# Autodesk Inventor assembly: Arm_Right
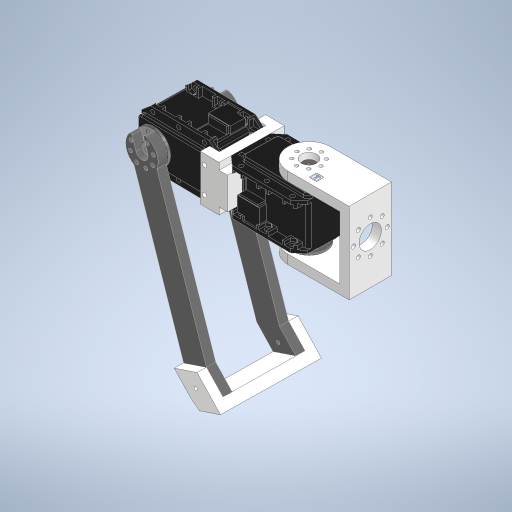
[picture p0: Inventor's stored thumbnail of the model, 512x512]
Saved by Autodesk Inventor 2024.3 (Build 283343000, 343)
## iProperties
Created: 2024-09-18
Part Number: Arm_Right
Document SubType Name: Assembly
Designer: 구지현
Author: 구지현
## Documents named in this file (9)
- C:\Users\구지현\Desktop\19th_intern_kdy_robot\부품\Upper_Body\Arm\Arm_Right.iam
- C:\Users\구지현\Desktop\19th_intern_kdy_robot\부품\Upper_Body\Arm\Hand.ipt
- C:\Users\구지현\Desktop\19th_intern_kdy_robot\부품\Upper_Body\Arm\Hand_Connection_Parts.ipt
- C:\Users\구지현\Desktop\19th_intern_kdy_robot\부품\Upper_Body\Arm\Middle_Arm_Fixing_Parts.ipt
- C:\Users\구지현\Documents\카카오톡 받은 파일\Hardware\ROBOTIS(Inventor 2024 ver.)\다이나믹셀\MX-28T_R+idle.ipt_MIR.iam
- C:\Users\구지현\Documents\카카오톡 받은 파일\Hardware\ROBOTIS(Inventor 2024 ver.)\혼\28Horn.ipt
- C:\Users\구지현\Desktop\19th_intern_kdy_robot\부품\Upper_Body\Arm\Shoulder_Fixing_Parts_Left_MIR.ipt
- C:\Users\구지현\Documents\카카오톡 받은 파일\Hardware\ROBOTIS(Inventor 2024 ver.)\다이나믹셀\MX-28T_R+idle.ipt_MIR_MIR.iam
- C:\Users\구지현\Documents\카카오톡 받은 파일\Hardware\ROBOTIS(Inventor 2024 ver.)\혼\28Horn_MIR.ipt
## Components (8 placed, 8 different names)
1. Hand:1 — 메이트:5, 메이트:6, 플러쉬:2, 삽입:8
2. Hand_Connection_Parts:1 — 플러쉬:2, 삽입:8
3. Middle_Arm_Fixing_Parts:1 — 메이트:1, 메이트:2, 메이트:3, 메이트:4, 삽입:6, 삽입:7
4. MX-28T_R+idle.ipt_MIR:2 [sub-assembly] — 삽입:2, 삽입:6, 삽입:7
5. 28Horn:2 — 삽입:2, 메이트:5, 메이트:6
6. Shoulder_Fixing_Parts_Left_MIR:1 — 플러쉬:1, 삽입:4
7. MX-28T_R+idle.ipt_MIR_MIR:1 [sub-assembly] — 삽입:5, 메이트:1, 메이트:2, 메이트:3, 메이트:4
8. 28Horn_MIR:1 — 삽입:4, 삽입:5
## Relationships (14: Insert 6, Mate 6, Flush 2)
- 삽입:2 [Insert]: MX-28T_R+idle.ipt_MIR:2 ↔ 28Horn:2
- 플러쉬:1 [Flush]: Shoulder_Fixing_Parts_Left_MIR:1
- 삽입:4 [Insert]: Shoulder_Fixing_Parts_Left_MIR:1 ↔ 28Horn_MIR:1
- 삽입:5 [Insert]: MX-28T_R+idle.ipt_MIR_MIR:1 ↔ 28Horn_MIR:1
- 메이트:1 [Mate] (0.1 mm): Middle_Arm_Fixing_Parts:1 ↔ MX-28T_R+idle.ipt_MIR_MIR:1
- 메이트:2 [Mate] (0.1 mm): Middle_Arm_Fixing_Parts:1 ↔ MX-28T_R+idle.ipt_MIR_MIR:1
- 메이트:3 [Mate]: Middle_Arm_Fixing_Parts:1 ↔ MX-28T_R+idle.ipt_MIR_MIR:1
- 메이트:4 [Mate]: Middle_Arm_Fixing_Parts:1 ↔ MX-28T_R+idle.ipt_MIR_MIR:1
- 삽입:6 [Insert]: Middle_Arm_Fixing_Parts:1 ↔ MX-28T_R+idle.ipt_MIR:2
- 삽입:7 [Insert]: Middle_Arm_Fixing_Parts:1 ↔ MX-28T_R+idle.ipt_MIR:2
- 메이트:5 [Mate]: Hand:1 ↔ 28Horn:2
- 메이트:6 [Mate]: Hand:1 ↔ 28Horn:2
- 플러쉬:2 [Flush]: Hand:1 ↔ Hand_Connection_Parts:1
- 삽입:8 [Insert]: Hand:1 ↔ Hand_Connection_Parts:1
